# Autodesk Inventor assembly: 2021 Drive
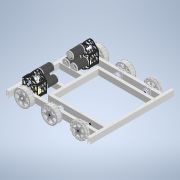
[picture p0: Inventor's stored thumbnail of the model, 180x180]
Saved by Autodesk Inventor 2022 (Build 260153000, 153)
## iProperties
Created: 2021-01-26
Part Number: 2021 Drive
Document SubType Name: Assembly
Designer: aidan
Author: aidan
## Documents named in this file (12)
- C:\Users\merky\OneDrive\Documents\t3-cad\CAD\2021 Specific Parts\2021 Drive.iam
- C:\Users\merky\OneDrive\Documents\t3-cad\CAD\VerseFrame 30in.ipt
- C:\Users\merky\OneDrive\Documents\t3-cad\CAD\2021 Specific Parts\VerseFrame 2021 28in Drive.ipt
- C:\Users\merky\OneDrive\Documents\t3-cad\CAD\WCP DS Gearbox.iam
- C:\Users\merky\OneDrive\Documents\t3-cad\CAD\Omni Wheel Assembly.iam
- C:\Users\merky\OneDrive\Documents\t3-cad\CAD\VersaBlock Assembly.iam
- C:\Users\merky\OneDrive\Documents\t3-cad\CAD\6in x 1.5in Wheel.iam
- C:\Users\merky\OneDrive\Documents\t3-cad\CAD\0.5in Hex Hub.ipt
- C:\Users\merky\OneDrive\Documents\t3-cad\CAD\Traction Wheel Assembly.iam
- C:\Users\merky\OneDrive\Documents\t3-cad\CAD\VerseFrame 16in.ipt
- C:\Users\merky\OneDrive\Documents\t3-cad\CAD\VerseFrame 20in.ipt
- C:\Users\merky\OneDrive\Documents\t3-cad\CAD\VerseFrame 8in.ipt
## Components (25 placed, 11 different names)
1. VerseFrame 30in:1 — Flush:2, Flush:5, Mate:1, Mate:37
2. VerseFrame 30in:2 — Flush:3, Flush:5, Mate:2, Flush:16, Flush:17, Mate:30, Flush:20, Flush:21, Mate:33
3. VerseFrame 2021 28in Drive:1 — Flush:1, Flush:2, Flush:4, Mate:1, Mate:2, Mate:3, Mate:4, Mate:8, Mate:21, Mate:23, Flush:16, Mate:34, Mate:38
4. VerseFrame 2021 28in Drive:2 — Flush:1, Flush:3, Flush:4, Mate:5, Mate:6, Mate:7, Mate:22, Mate:24, Flush:17, Mate:35, Mate:39
5. WCP DS Gearbox:1 [sub-assembly] — Mate:3, Mate:4, Mate:8, Mate:17, Mate:19
6. WCP DS Gearbox:2 [sub-assembly] — Mate:5, Mate:6, Mate:7, Mate:18, Mate:20
7. Omni Wheel Assembly:1 [sub-assembly] — Mate:27, Mate:28, Flush:19
8. Omni Wheel Assembly:2 [sub-assembly] — Mate:27, Flush:18, Mate:32
9. VersaBlock Assembly:1 [sub-assembly] — Flush:10, Flush:13, Mate:22, Flush:14, Mate:31
10. VersaBlock Assembly:2 [sub-assembly] — Flush:11, Flush:12, Flush:15, Mate:23, Mate:28, Mate:29, Mate:30, Mate:32
11. VersaBlock Assembly:3 [sub-assembly] — Flush:10, Mate:21, Flush:12, Flush:15, Mate:26, Mate:29
12. VersaBlock Assembly:4 [sub-assembly] — Flush:11, Flush:13, Flush:14, Mate:24
13. 6in x 1.5in Wheel:1 [sub-assembly] — Mate:9, Mate:10, Mate:11, Mate:12
14. 0.5in Hex Hub:1 — Flush:6, Flush:7, Mate:10, Mate:12
15. 0.5in Hex Hub:2 — Flush:6, Flush:7, Mate:9, Mate:11, Mate:17, Mate:19
16. 6in x 1.5in Wheel:2 [sub-assembly]
17. 0.5in Hex Hub:3 — Mate:20
18. 0.5in Hex Hub:4 — Mate:18
19. Traction Wheel Assembly:1 [sub-assembly] — Mate:25, Mate:26, Flush:19, Mate:31
20. Traction Wheel Assembly:2 [sub-assembly] — Mate:25, Flush:18
21. VerseFrame 20in:1 — Flush:20, Flush:22, Mate:33, Mate:34, Flush:23
22. VerseFrame 20in:2 — Flush:21, Flush:22, Mate:35, Mate:36, Flush:24
23. VerseFrame 16in:1 — Flush:23, Mate:36, Flush:24, Flush:27
24. VerseFrame 8in:1 — Flush:25, Flush:26, Mate:38
25. VerseFrame 8in:2 — Flush:25, Flush:26, Mate:37, Flush:27, Mate:39
## Relationships (66: Mate 39, Flush 27)
- Flush:1: VerseFrame 2021 28in Drive:1 ↔ VerseFrame 2021 28in Drive:2
- Flush:2: VerseFrame 30in:1 ↔ VerseFrame 2021 28in Drive:1
- Flush:3: VerseFrame 30in:2 ↔ VerseFrame 2021 28in Drive:2
- Flush:4: VerseFrame 2021 28in Drive:1 ↔ VerseFrame 2021 28in Drive:2
- Flush:5: VerseFrame 30in:1 ↔ VerseFrame 30in:2
- Mate:1: VerseFrame 30in:1 ↔ VerseFrame 2021 28in Drive:1
- Mate:2: VerseFrame 30in:2 ↔ VerseFrame 2021 28in Drive:1
- Mate:3: VerseFrame 2021 28in Drive:1 ↔ WCP DS Gearbox:1
- Mate:4: VerseFrame 2021 28in Drive:1 ↔ WCP DS Gearbox:1
- Mate:5: VerseFrame 2021 28in Drive:2 ↔ WCP DS Gearbox:2
- Mate:6: VerseFrame 2021 28in Drive:2 ↔ WCP DS Gearbox:2
- Mate:7: VerseFrame 2021 28in Drive:2 ↔ WCP DS Gearbox:2
- Mate:8: VerseFrame 2021 28in Drive:1 ↔ WCP DS Gearbox:1
- Flush:6: 0.5in Hex Hub:1 ↔ 0.5in Hex Hub:2
- Flush:7: 0.5in Hex Hub:1 ↔ 0.5in Hex Hub:2
- Mate:9: 6in x 1.5in Wheel:1 ↔ 0.5in Hex Hub:2
- Mate:10: 6in x 1.5in Wheel:1 ↔ 0.5in Hex Hub:1
- Mate:11: 6in x 1.5in Wheel:1 ↔ 0.5in Hex Hub:2
- Mate:12: 6in x 1.5in Wheel:1 ↔ 0.5in Hex Hub:1
- [Flush]: 0.5in Hex Hub:3 ↔ 0.5in Hex Hub:4
- [Flush]: 0.5in Hex Hub:3 ↔ 0.5in Hex Hub:4
- [Mate]: 6in x 1.5in Wheel:2 ↔ 0.5in Hex Hub:4
- [Mate]: 6in x 1.5in Wheel:2 ↔ 0.5in Hex Hub:3
- [Mate]: 6in x 1.5in Wheel:2 ↔ 0.5in Hex Hub:4
- [Mate]: 6in x 1.5in Wheel:2 ↔ 0.5in Hex Hub:3
- Mate:17: WCP DS Gearbox:1 ↔ 0.5in Hex Hub:2
- Mate:18: WCP DS Gearbox:2 ↔ 0.5in Hex Hub:4
- Mate:19: WCP DS Gearbox:1 ↔ 0.5in Hex Hub:2
- Mate:20: WCP DS Gearbox:2 ↔ 0.5in Hex Hub:3
- Flush:10: VersaBlock Assembly:1 ↔ VersaBlock Assembly:3
- Flush:11: VersaBlock Assembly:2 ↔ VersaBlock Assembly:4
- Mate:21: VerseFrame 2021 28in Drive:1 ↔ VersaBlock Assembly:3
- Flush:12: VersaBlock Assembly:2 ↔ VersaBlock Assembly:3
- Flush:13: VersaBlock Assembly:1 ↔ VersaBlock Assembly:4
- Mate:22: VerseFrame 2021 28in Drive:2 ↔ VersaBlock Assembly:1
- Flush:14: VersaBlock Assembly:1 ↔ VersaBlock Assembly:4
- Flush:15: VersaBlock Assembly:2 ↔ VersaBlock Assembly:3
- Mate:23: VerseFrame 2021 28in Drive:1 ↔ VersaBlock Assembly:2
- Mate:24: VerseFrame 2021 28in Drive:2 ↔ VersaBlock Assembly:4
- Mate:25: Traction Wheel Assembly:1 ↔ Traction Wheel Assembly:2
- Mate:26: VersaBlock Assembly:3 ↔ Traction Wheel Assembly:1
- Mate:27: Omni Wheel Assembly:1 ↔ Omni Wheel Assembly:2
- Mate:28: Omni Wheel Assembly:1 ↔ VersaBlock Assembly:2
- Flush:16 (-76.2 mm): VerseFrame 30in:2 ↔ VerseFrame 2021 28in Drive:1
- Flush:17 (76.2 mm): VerseFrame 30in:2 ↔ VerseFrame 2021 28in Drive:2
- Mate:29 (192.9384 mm): VersaBlock Assembly:2 ↔ VersaBlock Assembly:3
- Mate:30 (83.7692 mm): VerseFrame 30in:2 ↔ VersaBlock Assembly:2
- Flush:18: Omni Wheel Assembly:2 ↔ Traction Wheel Assembly:2
- Flush:19: Omni Wheel Assembly:1 ↔ Traction Wheel Assembly:1
- Mate:31: VersaBlock Assembly:1 ↔ Traction Wheel Assembly:1
- Mate:32: Omni Wheel Assembly:2 ↔ VersaBlock Assembly:2
- Flush:20: VerseFrame 30in:2 ↔ VerseFrame 20in:1
- Flush:21: VerseFrame 30in:2 ↔ VerseFrame 20in:2
- Flush:22: VerseFrame 20in:1 ↔ VerseFrame 20in:2
- Mate:33: VerseFrame 30in:2 ↔ VerseFrame 20in:1
- Mate:34 (50.8 mm): VerseFrame 2021 28in Drive:1 ↔ VerseFrame 20in:1
- Mate:35 (50.8 mm): VerseFrame 2021 28in Drive:2 ↔ VerseFrame 20in:2
- Flush:23: VerseFrame 20in:1 ↔ VerseFrame 16in:1
- Mate:36: VerseFrame 20in:2 ↔ VerseFrame 16in:1
- Flush:24: VerseFrame 20in:2 ↔ VerseFrame 16in:1
- Flush:25: VerseFrame 8in:1 ↔ VerseFrame 8in:2
- Flush:26: VerseFrame 8in:1 ↔ VerseFrame 8in:2
- Mate:37: VerseFrame 30in:1 ↔ VerseFrame 8in:2
- Flush:27: VerseFrame 16in:1 ↔ VerseFrame 8in:2
- Mate:38 (177.8 mm): VerseFrame 2021 28in Drive:1 ↔ VerseFrame 8in:1
- Mate:39 (177.8 mm): VerseFrame 2021 28in Drive:2 ↔ VerseFrame 8in:2
## Named parameters: d22_d16 = 0 mm, d23_d17 = 0 mm, d24_d18 = 0 mm, d25_d19 = 0 mm, d26_d20 = 0 mm, d27_d21 = 0 mm
